# Autodesk Inventor assembly: 01_Full_assembly
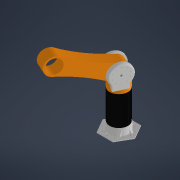
[picture p0: Inventor's stored thumbnail of the model, 180x180]
Saved by Autodesk Inventor 2022 (Build 260153000, 153)
## iProperties
Created: 2022-05-07
Part Number: 01_Full_assembly
Document SubType Name: Assembly
Designer: pzach
Author: pzach
## Documents named in this file (5)
- D:\GIT\Studia\Semestr4\MiSR\Robot\01_Full_assembly.iam
- D:\GIT\Studia\Semestr4\MiSR\Robot\01_Podstawa.ipt
- D:\GIT\Studia\Semestr4\MiSR\Robot\02_Bark.iam
- D:\GIT\Studia\Semestr4\MiSR\Robot\05_Bloczek.ipt
- D:\GIT\Studia\Semestr4\MiSR\Robot\04_Ramię-1.ipt
## Components (4 placed, 4 different names)
1. 01_Podstawa:1 — Insert:1
2. 02_Bark:1 [sub-assembly] — Insert:2, Insert:3
3. 05_Bloczek:1 — Insert:1, Angle:1, Insert:2
4. 04_Ramię-1:1 — Insert:3
## Relationships (4: Insert 3, Angle 1)
- Insert:1: 01_Podstawa:1 ↔ 05_Bloczek:1
- Angle:1 (0 deg): 05_Bloczek:1
- Insert:2: 02_Bark:1 ↔ 05_Bloczek:1
- Insert:3: 02_Bark:1 ↔ 04_Ramię-1:1
